# Autodesk Inventor assembly: konsola
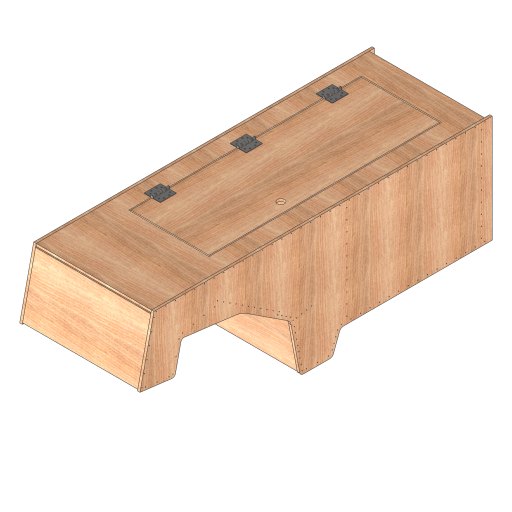
[picture p0: Inventor's stored thumbnail of the model, 512x512]
Saved by Autodesk Inventor 2023.2 (Build 272271030, 271C)
## iProperties
RuleStatus: InUse
Created: 2022-11-02
Part Number: konsola
Document SubType Name: Assembly
Designer: GUT
Author: GUT
## Documents named in this file (24)
- C:\Users\GUT\Desktop\konsola\projekt\konsola.iam
- C:\Users\GUT\Desktop\konsola\projekt\CUT PART A-01.ipt
- C:\Users\GUT\Desktop\konsola\projekt\CUT PART B-01.ipt
- C:\Users\GUT\Desktop\konsola\projekt\CUT PART C-01.ipt
- C:\Users\GUT\Desktop\konsola\projekt\CUT PART D-01.ipt
- C:\Users\GUT\Desktop\konsola\projekt\CUT PART G-01.ipt
- C:\Users\GUT\Desktop\konsola\projekt\CUT PART H-01.ipt
- C:\Users\GUT\Desktop\konsola\projekt\CUT PART I-01.ipt
- C:\Users\GUT\Desktop\konsola\projekt\CUT PART J-01.ipt
- C:\Users\GUT\Desktop\konsola\projekt\CUT PART K-01.ipt
- C:\Users\GUT\Desktop\konsola\projekt\monitor.ipt
- C:\Users\GUT\Desktop\konsola\projekt\CUT PART N-01.ipt
- C:\Users\GUT\Desktop\konsola\projekt\CUT PART O-01.ipt
- C:\Users\GUT\Desktop\konsola\projekt\CUT PART P-01.ipt
- C:\Users\GUT\Desktop\konsola\projekt\CUT PART R-01.ipt
- C:\Users\GUT\Desktop\konsola\projekt\zawias-prawy.ipt
- C:\Users\GUT\Desktop\konsola\projekt\zawias-lewy.ipt
- C:\Users\GUT\Desktop\konsola\projekt\trzpien.ipt
- C:\Users\GUT\Desktop\konsola\projekt\konsola\AIP\FEA\e5rbyew00.fins
- C:\Users\GUT\Desktop\konsola\projekt\konsola\AIP\FEA\e5rbyew00.fsat
- C:\Users\GUT\Desktop\konsola\projekt\konsola\AIP\FEA\e5rbyew00.ftes
- C:\Users\GUT\Desktop\konsola\projekt\konsola\AIP\FEA\e5rbyew00.fwiz
- C:\Users\GUT\Desktop\konsola\projekt\konsola\AIP\FEA\e5rbyewao.fmsh
- C:\Users\GUT\Desktop\konsola\projekt\konsola\AIP\FEA\e5rbyewap.fres
## Components (28 placed, 17 different names)
1. CUT PART A-01:1 — Mate:2, Flush:3, Flush:4, Mate:3, Flush:5, Mate:4, Flush:6, Flush:7, Flush:8, Mate:6, Flush:10, Mate:7, Flush:12, Mate:21, Mate:34, Mate:39, Mate:40
2. CUT PART A-01:2 — Mate:5, Flush:8, Flush:12, Mate:10, Flush:13, Mate:11, Mate:12, Flush:14, Mate:13, Mate:17, Mate:18, Angle:3, Flush:15, Mate:26, Mate:29, Flush:19, Mate:31, Flush:20, Mate:36
3. CUT PART B-01:1 — Mate:6, Flush:10, Mate:7, Mate:32
4. CUT PART C-01:1 — Mate:10, Flush:13, Mate:11, Mate:19, Angle:4
5. CUT PART D-01:1 — Mate:21, Flush:15, Mate:28
6. CUT PART G-01:1 — Mate:2, Flush:3, Flush:4, Mate:5, Flush:26, Mate:42, Mate:43, Mate:56, Mate:57, Mate:58, Mate:59, Mate:60, Mate:61
7. CUT PART H-01:1 — Mate:18, Mate:19, Angle:4
8. CUT PART I-01:1 — Mate:4, Flush:6, Flush:7, Mate:30, Mate:33, Mate:35, Flush:21
9. CUT PART J-01:1 — Mate:3, Flush:5, Mate:33
10. CUT PART J-01:2 — Mate:34, Mate:35, Flush:21
11. CUT PART K-01:1 — Mate:12, Flush:14, Mate:13, Mate:20, Mate:28, Mate:41, Flush:24
12. CUT PART N-01:1 — Mate:29, Flush:19, Mate:30
13. CUT PART N-01:2 — Mate:40, Mate:41, Flush:24
14. CUT PART N-01:3 — Mate:17, Mate:20, Angle:3, Mate:27
15. CUT PART O-01:1 — Mate:31, Flush:20, Mate:32
16. CUT PART P-01:1 — Mate:38, Mate:39, Flush:22, Flush:25
17. CUT PART P-01:2 — Mate:36, Mate:37, Flush:22
18. CUT PART R-01:1 — Flush:26, Mate:42, Mate:43, Flush:27, Flush:28, Flush:29, Mate:62, Mate:63, Mate:64
19. monitor:1 — Mate:26, Mate:27, Mate:37, Mate:38, Flush:25
20. zawias-prawy:1 — Mate:44, Mate:45, Mate:56, Flush:28, Mate:59
21. zawias-lewy:1 — Mate:44, Mate:45, Mate:46, Mate:47, Mate:63
22. trzpien:1 — Mate:46, Mate:47
23. zawias-prawy:2 — Mate:58, Flush:29, Mate:61
24. zawias-lewy:2 — Mate:64
25. trzpien:2
26. zawias-prawy:3 — Mate:57, Flush:27, Mate:60
27. zawias-lewy:3 — Mate:62
28. trzpien:3
## Relationships (77: Mate 54, Flush 21, Angle 2)
- Mate:2: CUT PART A-01:1 ↔ CUT PART G-01:1
- Flush:3: CUT PART A-01:1 ↔ CUT PART G-01:1
- Flush:4 (-25 mm): CUT PART A-01:1 ↔ CUT PART G-01:1
- Mate:3: CUT PART A-01:1 ↔ CUT PART J-01:1
- Flush:5 (45 mm): CUT PART A-01:1 ↔ CUT PART J-01:1
- Mate:4: CUT PART A-01:1 ↔ CUT PART I-01:1
- Flush:6 (6 mm): CUT PART A-01:1 ↔ CUT PART I-01:1
- Flush:7 (25 mm): CUT PART A-01:1 ↔ CUT PART I-01:1
- Mate:5: CUT PART A-01:2 ↔ CUT PART G-01:1
- Flush:8: CUT PART A-01:1 ↔ CUT PART A-01:2
- Mate:6: CUT PART A-01:1 ↔ CUT PART B-01:1
- Flush:10: CUT PART A-01:1 ↔ CUT PART B-01:1
- Mate:7 (-6 mm): CUT PART A-01:1 ↔ CUT PART B-01:1
- Flush:12: CUT PART A-01:1 ↔ CUT PART A-01:2
- Mate:10: CUT PART A-01:2 ↔ CUT PART C-01:1
- Flush:13 (6 mm): CUT PART A-01:2 ↔ CUT PART C-01:1
- Mate:11 (6 mm): CUT PART A-01:2 ↔ CUT PART C-01:1
- Mate:12: CUT PART A-01:2 ↔ CUT PART K-01:1
- Flush:14 (6 mm): CUT PART A-01:2 ↔ CUT PART K-01:1
- Mate:13 (-6 mm): CUT PART A-01:2 ↔ CUT PART K-01:1
- Mate:17: CUT PART A-01:2 ↔ CUT PART N-01:3
- Mate:18: CUT PART A-01:2 ↔ CUT PART H-01:1
- Mate:19: CUT PART C-01:1 ↔ CUT PART H-01:1
- Mate:20: CUT PART K-01:1 ↔ CUT PART N-01:3
- Angle:3 (0 deg): CUT PART A-01:2 ↔ CUT PART N-01:3
- Mate:21: CUT PART A-01:1 ↔ CUT PART D-01:1
- Flush:15 (8 mm): CUT PART A-01:2 ↔ CUT PART D-01:1
- Mate:26 (0.5 mm): CUT PART A-01:2 ↔ monitor:1
- Mate:27 (3 mm): CUT PART N-01:3 ↔ monitor:1
- Angle:4 (66 deg): CUT PART C-01:1 ↔ CUT PART H-01:1
- Mate:28 (2 mm): CUT PART D-01:1 ↔ CUT PART K-01:1
- Mate:29: CUT PART A-01:2 ↔ CUT PART N-01:1
- Flush:19 (6 mm): CUT PART A-01:2 ↔ CUT PART N-01:1
- Mate:30 (1 mm): CUT PART I-01:1 ↔ CUT PART N-01:1
- Mate:31: CUT PART A-01:2 ↔ CUT PART O-01:1
- Flush:20 (6 mm): CUT PART A-01:2 ↔ CUT PART O-01:1
- Mate:32 (1.5 mm): CUT PART B-01:1 ↔ CUT PART O-01:1
- Mate:33 (5 mm): CUT PART I-01:1 ↔ CUT PART J-01:1
- Mate:34: CUT PART A-01:1 ↔ CUT PART J-01:2
- Mate:35 (5 mm): CUT PART I-01:1 ↔ CUT PART J-01:2
- Flush:21 (-30 mm): CUT PART I-01:1 ↔ CUT PART J-01:2
- Mate:36: CUT PART A-01:2 ↔ CUT PART P-01:2
- Mate:37: CUT PART P-01:2 ↔ monitor:1
- Mate:38: CUT PART P-01:1 ↔ monitor:1
- Mate:39: CUT PART A-01:1 ↔ CUT PART P-01:1
- Flush:22: CUT PART P-01:1 ↔ CUT PART P-01:2
- Mate:40: CUT PART A-01:1 ↔ CUT PART N-01:2
- Mate:41: CUT PART K-01:1 ↔ CUT PART N-01:2
- Flush:24 (5 mm): CUT PART K-01:1 ↔ CUT PART N-01:2
- Flush:25 (-25.5 mm): CUT PART P-01:1 ↔ monitor:1
- Flush:26: CUT PART G-01:1 ↔ CUT PART R-01:1
- Mate:42 (5 mm): CUT PART G-01:1 ↔ CUT PART R-01:1
- Mate:43 (5 mm): CUT PART G-01:1 ↔ CUT PART R-01:1
- Mate:44: zawias-prawy:1 ↔ zawias-lewy:1
- Mate:45: zawias-prawy:1 ↔ zawias-lewy:1
- Mate:46: zawias-lewy:1 ↔ trzpien:1
- Mate:47: zawias-lewy:1 ↔ trzpien:1
- [Mate]: zawias-prawy:2 ↔ zawias-lewy:2
- [Mate]: zawias-prawy:2 ↔ zawias-lewy:2
- [Mate]: zawias-lewy:2 ↔ trzpien:2
- [Mate]: zawias-lewy:2 ↔ trzpien:2
- [Mate]: zawias-prawy:3 ↔ zawias-lewy:3
- [Mate]: zawias-prawy:3 ↔ zawias-lewy:3
- [Mate]: zawias-lewy:3 ↔ trzpien:3
- [Mate]: zawias-lewy:3 ↔ trzpien:3
- Mate:56: CUT PART G-01:1 ↔ zawias-prawy:1
- Mate:57: CUT PART G-01:1 ↔ zawias-prawy:3
- Mate:58: CUT PART G-01:1 ↔ zawias-prawy:2
- Flush:27 (506.9 mm): CUT PART R-01:1 ↔ zawias-prawy:3
- Flush:28 (100 mm): CUT PART R-01:1 ↔ zawias-prawy:1
- Flush:29 (100 mm): CUT PART R-01:1 ↔ zawias-prawy:2
- Mate:59 (-32.1 mm): CUT PART G-01:1 ↔ zawias-prawy:1
- Mate:60 (-32.1 mm): CUT PART G-01:1 ↔ zawias-prawy:3
- Mate:61 (-32.1 mm): CUT PART G-01:1 ↔ zawias-prawy:2
- Mate:62: CUT PART R-01:1 ↔ zawias-lewy:3
- Mate:63: CUT PART R-01:1 ↔ zawias-lewy:1
- Mate:64: CUT PART R-01:1 ↔ zawias-lewy:2
## Named parameters: width = 545 mm, thickness = 12 mm, sa_0 = 981, odl = 5 mm, lenJ = 464 mm, lenB = 285 mm, lenC = 153 mm, lenD = 125 mm, lenG = 1575 mm, lenH = 175 mm, lenI = 699 mm, lenK = 251 mm, lenN = 93 mm, lenO = 133 mm, lenP = 370 mm, d80_d76 = 0 mm, d81_d77 = 0 mm, d82_d78 = 0 mm, d83_d79 = 0 mm, d84_d76 = 0 mm, d85_d77 = 0 mm, d86_d78 = 0 mm, d87_d79 = 0 mm, lenR = 1090 mm, inter = 100 mm, l_z = -32.1 mm
note: some values were not read from the file. Shown as the stored number, unit unknown: "sa_0".
